# Autodesk Inventor assembly: FB32_FH23_SlipRing
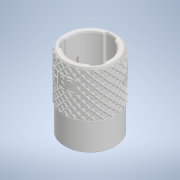
[picture p0: Inventor's stored thumbnail of the model, 180x180]
Saved by Autodesk Inventor 2020.2 (Build 242310000, 310)
## iProperties
Created: 2020-03-13
Part Number: FB32_FH23_SlipRing
Document SubType Name: Assembly
Designer: Rudi
Author: Rudi
## Documents named in this file (4)
- C:\Users\Rudi\Documents\Privat\Rudi\Hobbyhimmel\Klar Schiff\CAD-Modelle-Fertigungsdaten\3D-Modelle\osVac\Bayonet_V1.1\FB32_FH23_SlipRing.iam
- C:\Users\Rudi\Documents\Privat\Rudi\Hobbyhimmel\Klar Schiff\CAD-Modelle-Fertigungsdaten\3D-Modelle\osVac\Bayonet_V1.1\FB32_Base.ipt
- C:\Users\Rudi\Documents\Privat\Rudi\Hobbyhimmel\Klar Schiff\CAD-Modelle-Fertigungsdaten\3D-Modelle\osVac\Bayonet_V1.1\Drehkupplung.ipt
- C:\Users\Rudi\Documents\Privat\Rudi\Hobbyhimmel\Klar Schiff\CAD-Modelle-Fertigungsdaten\3D-Modelle\osVac\Bayonet_V1.1\FH32_Base.ipt
## Components (3 placed, 3 different names)
1. FB32_Base:1 — Passend:5, Passend:6, Fluchtend:1
2. Drehkupplung:1 — Passend:3, Passend:4, Passend:5, Fluchtend:1
3. FH32_Base:1 — Passend:3, Passend:4, Passend:6
## Relationships (5: Mate 4, Flush 1)
- Passend:3 [Mate]: Drehkupplung:1 ↔ FH32_Base:1
- Passend:4 [Mate]: Drehkupplung:1 ↔ FH32_Base:1
- Passend:5 [Mate]: FB32_Base:1 ↔ Drehkupplung:1
- Passend:6 [Mate]: FB32_Base:1 ↔ FH32_Base:1
- Fluchtend:1 [Flush]: FB32_Base:1 ↔ Drehkupplung:1
